# Autodesk Inventor assembly: shaftSealAssembly2
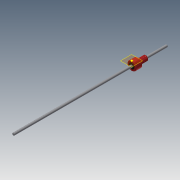
[picture p0: Inventor's stored thumbnail of the model, 180x180]
Saved by Autodesk Inventor 2018 (Build 220112000, 112)
## iProperties
Created: 2020-03-03
Part Number: shaftSealAssembly2
Document SubType Name: Assembly
Designer: anirudh.bali
Author: anirudh.bali
## Documents named in this file (6)
- D:\Silicon Sharks\2019-2020\servoBox\shaftSeal\shaftSealAssembly2.iam
- D:\Silicon Sharks\2019-2020\servoBox\shaftSeal\6362K111_WATER-RESISTANT DRY-RUNNING SLEEVE BEARING.ipt
- D:\Silicon Sharks\2019-2020\servoBox\shaftSeal\6362K211_WATER-RESISTANT DRY-RUNNING SLEEVE BEARING.ipt
- D:\Silicon Sharks\2019-2020\servoBox\shaftSeal\cupORing.ipt
- D:\Silicon Sharks\2019-2020\servoBox\shaftSeal\1257K530_MINIATURE 303 STAINLESS STEEL DRIVE SHAFT.ipt
- D:\Silicon Sharks\2019-2020\servoBox\shaftSeal\shaftSealBulkhead2.ipt
## Components (7 placed, 5 different names)
1. 6362K111_WATER-RESISTANT DRY-RUNNING SLEEVE BEARING:1 — Mate:9, Mate:14
2. 6362K211_WATER-RESISTANT DRY-RUNNING SLEEVE BEARING:1 — Mate:1, Mate:2, Mate:3, Mate:10
3. cupORing:1 — Mate:3, Mate:5, Mate:10, Mate:11
4. 6362K111_WATER-RESISTANT DRY-RUNNING SLEEVE BEARING:2 — Mate:5, Mate:7, Mate:12
5. cupORing:2 — Mate:7, Mate:9, Mate:13
6. 1257K530_MINIATURE 303 STAINLESS STEEL DRIVE SHAFT:1 — Mate:15, Mate:16
7. shaftSealBulkhead2:1 — Mate:1, Mate:2, Mate:11, Mate:12, Mate:13, Mate:14, Mate:15, Mate:16
## Relationships (13: Mate 13)
- Mate:1: 6362K211_WATER-RESISTANT DRY-RUNNING SLEEVE BEARING:1 ↔ shaftSealBulkhead2:1
- Mate:2: 6362K211_WATER-RESISTANT DRY-RUNNING SLEEVE BEARING:1 ↔ shaftSealBulkhead2:1
- Mate:3: 6362K211_WATER-RESISTANT DRY-RUNNING SLEEVE BEARING:1 ↔ cupORing:1
- Mate:5: cupORing:1 ↔ 6362K111_WATER-RESISTANT DRY-RUNNING SLEEVE BEARING:2
- Mate:7: 6362K111_WATER-RESISTANT DRY-RUNNING SLEEVE BEARING:2 ↔ cupORing:2
- Mate:9: 6362K111_WATER-RESISTANT DRY-RUNNING SLEEVE BEARING:1 ↔ cupORing:2
- Mate:10: 6362K211_WATER-RESISTANT DRY-RUNNING SLEEVE BEARING:1 ↔ cupORing:1
- Mate:11: cupORing:1 ↔ shaftSealBulkhead2:1
- Mate:12: 6362K111_WATER-RESISTANT DRY-RUNNING SLEEVE BEARING:2 ↔ shaftSealBulkhead2:1
- Mate:13: cupORing:2 ↔ shaftSealBulkhead2:1
- Mate:14: 6362K111_WATER-RESISTANT DRY-RUNNING SLEEVE BEARING:1 ↔ shaftSealBulkhead2:1
- Mate:15: 1257K530_MINIATURE 303 STAINLESS STEEL DRIVE SHAFT:1 ↔ shaftSealBulkhead2:1
- Mate:16 (-69.85 mm): 1257K530_MINIATURE 303 STAINLESS STEEL DRIVE SHAFT:1 ↔ shaftSealBulkhead2:1
